# Autodesk Inventor assembly: MAQUINADO CAVIDAD 2
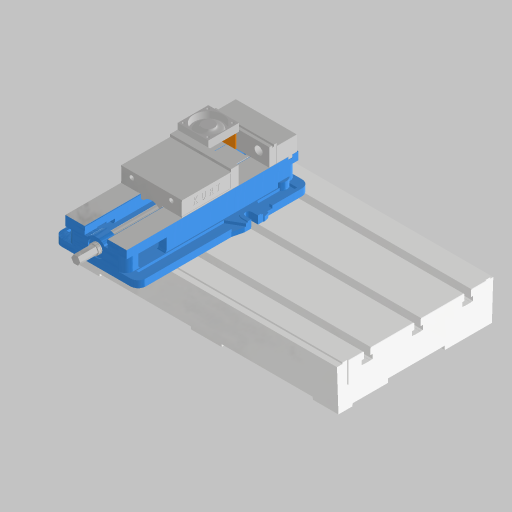
[picture p0: Inventor's stored thumbnail of the model, 512x512]
Saved by Autodesk Inventor 2024 (Build 280153000, 153)
## iProperties
Created: 2023-02-15
Part Number: MAQUINADO CAVIDAD 2
Document SubType Name: Assembly
Designer: rodar
Author: rodar
## Documents named in this file (4)
- G:\Unidades compartidas\Cursos de Ingeniería Mecánica UVG\Cursos IMXXX\IM3027 Introducción a Diseño y Manufactura CAD CAM\Clases - 2do semestre 2023\S7C1 - INVENTOR CAM\7 - MAQUINADO CAVIDAD 2.iam
- G:\Unidades compartidas\Cursos de Ingeniería Mecánica UVG\Cursos IMXXX\IM3027 Introducción a Diseño y Manufactura CAD CAM\Clases - 2do semestre 2023\S7C1 - INVENTOR CAM\Fixture\VF1 TABLE + FLEX_KURT D688.iam
- G:\Unidades compartidas\Cursos de Ingeniería Mecánica UVG\Cursos IMXXX\IM3027 Introducción a Diseño y Manufactura CAD CAM\Clases - 2do semestre 2023\S7C1 - INVENTOR CAM\6 - CAVIDAD MATERIAL 2.ipt
- G:\Unidades compartidas\Cursos de Ingeniería Mecánica UVG\Cursos IMXXX\IM3027 Introducción a Diseño y Manufactura CAD CAM\Clases - 2do semestre 2023\S7C1 - INVENTOR CAM\Fixture\ALZA MAQUINADO.ipt
## Components (4 placed, 3 different names)
1. VF1 TABLE + FLEX_KURT D688:1 [sub-assembly] — Mate:1, Mate:2, Flush:1, Mate:3, Mate:4, Mate:5, Flush:2
2. 6 - CAVIDAD MATERIAL 2:1 — Mate:1, Mate:2, Flush:1, Mate:3
3. ALZA MAQUINADO:1 — Mate:4, Mate:5, Flush:2
4. ALZA MAQUINADO:2
## Component patterns: (2 elements, first: ALZA MAQUINADO:1)
## Relationships (7: Mate 5, Flush 2)
- Mate:1 (40 mm): VF1 TABLE + FLEX_KURT D688:1 ↔ 6 - CAVIDAD MATERIAL 2:1
- Mate:2: VF1 TABLE + FLEX_KURT D688:1 ↔ 6 - CAVIDAD MATERIAL 2:1
- Flush:1: VF1 TABLE + FLEX_KURT D688:1 ↔ 6 - CAVIDAD MATERIAL 2:1
- Mate:3: VF1 TABLE + FLEX_KURT D688:1 ↔ 6 - CAVIDAD MATERIAL 2:1
- Mate:4: VF1 TABLE + FLEX_KURT D688:1 ↔ ALZA MAQUINADO:1
- Mate:5: VF1 TABLE + FLEX_KURT D688:1 ↔ ALZA MAQUINADO:1
- Flush:2: VF1 TABLE + FLEX_KURT D688:1 ↔ ALZA MAQUINADO:1
